# Autodesk Inventor assembly: ASY Лестница
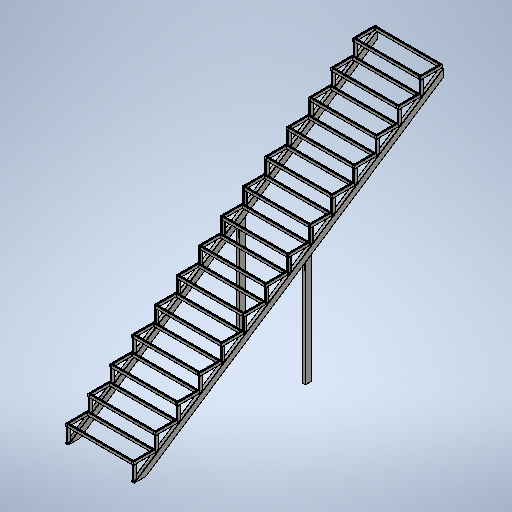
[picture p0: Inventor's stored thumbnail of the model, 512x512]
Saved by Autodesk Inventor 2025 (Build 290162010, 162A)
## iProperties
Created: 2025-01-21
Part Number: ASY Лестница
Document SubType Name: Assembly
Designer: pokla
Author: pokla
## Documents named in this file (4)
- C:\Users\pokla\Documents\Inventor\NDM-VOS_powder_hopper\ASY Лестница.iam
- C:\Users\pokla\Documents\Inventor\NDM-VOS_powder_hopper\ASY_Ступень.iam
- C:\Users\pokla\Documents\Inventor\NDM-VOS_powder_hopper\ISO 4019 - 80x40x2 - 4381,295.ipt
- C:\Users\pokla\Documents\Inventor\NDM-VOS_powder_hopper\ISO 4019 - 80x40x2 - 1300.ipt
## Components (18 placed, 3 different names)
1. ISO 4019 - 80x40x2 - 4381,295:1 — Rigid:1, Flush:1, Mate:1
2. ISO 4019 - 80x40x2 - 4381,295:2 — Rigid:2
3. ISO 4019 - 80x40x2 - 1300:1 — Flush:1, Mate:1, Rigid:3
4. ISO 4019 - 80x40x2 - 1300:2 — Rigid:3
5. ASY_Ступень:1 [sub-assembly]
6. ASY_Ступень:2 [sub-assembly]
7. ASY_Ступень:3 [sub-assembly]
8. ASY_Ступень:4 [sub-assembly]
9. ASY_Ступень:5 [sub-assembly]
10. ASY_Ступень:6 [sub-assembly]
11. ASY_Ступень:7 [sub-assembly]
12. ASY_Ступень:8 [sub-assembly]
13. ASY_Ступень:9 [sub-assembly]
14. ASY_Ступень:10 [sub-assembly]
15. ASY_Ступень:11 [sub-assembly]
16. ASY_Ступень:12 [sub-assembly]
17. ASY_Ступень:13 [sub-assembly]
18. ASY_Ступень:14 [sub-assembly] — Rigid:1, Rigid:2
## Component patterns: (14 elements, first: ASY_Ступень:1)
## Relationships (5: WeldJoint 3, Flush 1, Mate 1)
- Rigid:1 [WeldJoint]: ISO 4019 - 80x40x2 - 4381,295:1 ↔ ASY_Ступень:14
- Rigid:2 [WeldJoint]: ISO 4019 - 80x40x2 - 4381,295:2 ↔ ASY_Ступень:14
- Flush:1: ISO 4019 - 80x40x2 - 4381,295:1 ↔ ISO 4019 - 80x40x2 - 1300:1
- Mate:1: ISO 4019 - 80x40x2 - 4381,295:1 ↔ ISO 4019 - 80x40x2 - 1300:1
- Rigid:3 [WeldJoint] (740 mm): ISO 4019 - 80x40x2 - 1300:1 ↔ ISO 4019 - 80x40x2 - 1300:2
